# Autodesk Inventor assembly: RasPiArm基板
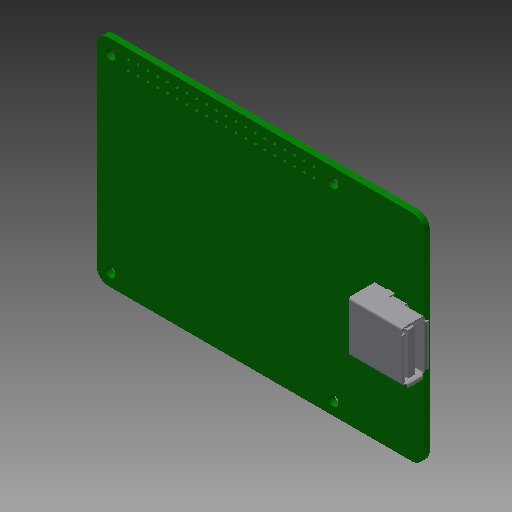
[picture p0: Inventor's stored thumbnail of the model, 512x512]
Saved by Autodesk Inventor 2017 (Build 210142000, 142)
## iProperties
Created: 2016-08-22
Part Number: RasPiArm基板
Material: 一般
Document SubType Name: Assembly
Designer: NN
Mass: 13.4034 g
Surface Area: 117.858 cm^2
Volume: 8.14168 cm^3
Density: 1.64627 g/cm^3
Author: NN
## Documents named in this file (3)
- C:\Users\karaage\Downloads\RaspberryPiGibbon-master\RaspberryPiGibbon-master\CAD\汎用パーツ\RasPiArm基板\RasPiArm基板.iam
- C:\Users\karaage\Downloads\RaspberryPiGibbon-master\RaspberryPiGibbon-master\CAD\汎用パーツ\RasPiArm基板\14377.ipt
- C:\Users\karaage\Downloads\RaspberryPiGibbon-master\RaspberryPiGibbon-master\CAD\汎用パーツ\RasPiArm基板\RasPiArm基板.ipt
## Components (2 placed, 2 different names)
1. 14377:1 — メイト:1, フラッシュ:1, フラッシュ:2
2. RasPiArm基板:1 — メイト:1, フラッシュ:1, フラッシュ:2
## Relationships (3: Flush 2, Mate 1)
- メイト:1 [Mate]: 14377:1 ↔ RasPiArm基板:1
- フラッシュ:1 [Flush] (-1.9 mm): 14377:1 ↔ RasPiArm基板:1
- フラッシュ:2 [Flush] (-20.4 mm): 14377:1 ↔ RasPiArm基板:1
